# Autodesk Inventor assembly: BottomPart
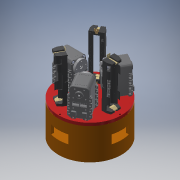
[picture p0: Inventor's stored thumbnail of the model, 180x180]
Saved by Autodesk Inventor 2019 (Build 230136000, 136)
## iProperties
Created: 2022-07-05
Part Number: BottomPart
Document SubType Name: Assembly
Designer: zreik
Author: zreik
## Documents named in this file (5)
- D:\Documents\HIAST\4th year\4th Year Project\Design\BottomPart.iam
- D:\Documents\HIAST\4th year\4th Year Project\Design\Base.ipt
- D:\Documents\HIAST\4th year\4th Year Project\Design\Cover.ipt
- D:\Documents\HIAST\4th year\4th Year Project\Design\AX-12A\AX-12A.iam
- D:\Documents\HIAST\4th year\4th Year Project\Design\BatteryHolder.ipt
## Components (8 placed, 4 different names)
1. Base:1 — Mate:1, Mate:2, Mate:3, Mate:11, Mate:12, Mate:13
2. Cover:1 — Mate:1, Mate:2, Mate:3, Mate:6, Mate:14
3. AX-12A:1 [sub-assembly] — Mate:6, Flush:1, Flush:2, Angle:1
4. AX-12A:2 [sub-assembly]
5. AX-12A:3 [sub-assembly]
6. BatteryHolder:1 — Mate:14, Angle:1
7. BatteryHolder:2
8. BatteryHolder:3
## Component patterns: (3 elements, first: AX-12A:1), (3 elements, first: BatteryHolder:1)
## Relationships (11: Mate 8, Flush 2, Angle 1)
- Mate:1: Base:1 ↔ Cover:1
- Mate:2: Base:1 ↔ Cover:1
- Mate:3: Base:1 ↔ Cover:1
- Mate:6: Cover:1 ↔ AX-12A:1
- Mate:11: Base:1
- Mate:12: Base:1
- Mate:13: Base:1
- Flush:1 (15 mm): AX-12A:1
- Flush:2: AX-12A:1
- Mate:14: Cover:1 ↔ BatteryHolder:1
- Angle:1 (60 deg): AX-12A:1 ↔ BatteryHolder:1
